# Autodesk Inventor assembly: TMH4A - 2 V2
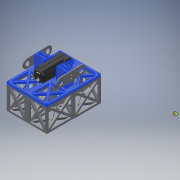
[picture p0: Inventor's stored thumbnail of the model, 180x180]
Saved by Autodesk Inventor 2019 (Build 230136000, 136)
## iProperties
Created: 2019-01-06
Part Number: TMH4A - 2 V2
Document SubType Name: Assembly
Designer: ashle
Author: ashle
## Documents named in this file (5)
- C:\Users\ashle\OneDrive\Desktop\FTC repositories\design\inventor\2018-2019\Tape Measure Holder\4 Tape Measure Holder\TMH4A - 2 V2.iam
- C:\Users\ashle\OneDrive\Desktop\FTC repositories\design\inventor\2018-2019\Tape Measure Holder\4 Tape Measure Holder\4 Tape Measure Holder 2 Lid.ipt
- C:\Users\ashle\OneDrive\Desktop\FTC repositories\design\inventor\Imported Components\REV\Motors and Servos\REVCoreHexMotor.ipt
- C:\Users\ashle\OneDrive\Desktop\FTC repositories\design\inventor\2018-2019\Tape Measure Holder\4 Tape Measure Holder\Version One\4 Tape Measures Holder 2.ipt
- C:\Users\ashle\OneDrive\Desktop\FTC repositories\design\inventor\2018-2019\Tape Measure Holder\4 Tape Measure Holder\Side Attatchment V2.ipt
## Components (5 placed, 4 different names)
1. 4 Tape Measure Holder 2 Lid:1 — Insert:1, Insert:2, Insert:3, Insert:4, Insert:5, Insert:6, Insert:7, Insert:8, Insert:9, Insert:10
2. REVCoreHexMotor:1 — Insert:5, Insert:6
3. 4 Tape Measures Holder 2:1 — Insert:1, Insert:2, Insert:3, Insert:4
4. Side Attatchment V2:1 — Insert:8, Insert:10
5. Side Attatchment V2:2 — Insert:7, Insert:9
## Relationships (10: Insert 10)
- Insert:1: 4 Tape Measure Holder 2 Lid:1 ↔ 4 Tape Measures Holder 2:1
- Insert:2: 4 Tape Measure Holder 2 Lid:1 ↔ 4 Tape Measures Holder 2:1
- Insert:3: 4 Tape Measure Holder 2 Lid:1 ↔ 4 Tape Measures Holder 2:1
- Insert:4: 4 Tape Measure Holder 2 Lid:1 ↔ 4 Tape Measures Holder 2:1
- Insert:5: 4 Tape Measure Holder 2 Lid:1 ↔ REVCoreHexMotor:1
- Insert:6: 4 Tape Measure Holder 2 Lid:1 ↔ REVCoreHexMotor:1
- Insert:7: 4 Tape Measure Holder 2 Lid:1 ↔ Side Attatchment V2:2
- Insert:8: 4 Tape Measure Holder 2 Lid:1 ↔ Side Attatchment V2:1
- Insert:9: 4 Tape Measure Holder 2 Lid:1 ↔ Side Attatchment V2:2
- Insert:10: 4 Tape Measure Holder 2 Lid:1 ↔ Side Attatchment V2:1
